# Autodesk Inventor assembly: SBGSMA6200ZZ-20
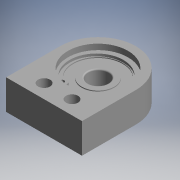
[picture p0: Inventor's stored thumbnail of the model, 180x180]
Saved by Autodesk Inventor 2017.3 (Build 213256000, 256)
## iProperties
Category: PARTsolutions
Company: MISUMI
Part Number: SBGSMA6200ZZ-20
Catalog Web Link: www.cadenas.de
Description: BGSMA, BGSMAB, SBGSMA-Bearing with Housings - Front Installation Type
Vendor: MISUMI
Document SubType Name: Assembly
Designer: partserver
Manufacturer: MISUMI
Mass: 18.5202 g
Surface Area: 96.0337 cm^2
Volume: 18.5202 cm^3
Density: 1 g/cm^3
Title: SBGSMA6200ZZ-20
Author: Cadenas PARTsolutions
Comments: Bearing with Housings - Front Installation Type
PSOL_IDENT_0: {$CADENAS_DATA\23d-libs\misumi\metric\12_bearing_holders\bgsma_asmtab.prj},222 {VTYP=3D},{STYP=ASSTA
PSOL_IDENT_1: B},{NB=SBGSMA6200ZZ-20},{LINA=SBGSMA6200ZZ-20},{NN=BGSMA, BGSMAB, SBGSMA},{DATE=09.09.2019 15:26:56}
PSOL_IDENT_2: ,{GEOMDATE=13.07.2015 10:17:28},{VERSION=},{LINEID=30},{WBVAR=MATB,STH,SEAL,HH,ALT1},{WBNUMERIC=HH}
PSOL_IDENT_3: {NB=SBGSMA6200ZZ-20},{LINA=SBGSMA6200ZZ-20},{KT=DUMMY},{PN=SBGSMA6200ZZ-20},{TYPE=SBGSMA},{MATB=STS
PSOL_IDENT_4: },{MATBALG= 'ST','Steel','STS','Stainless Steel' },{STH=},{STHALG= '','-' },{ARR=304 Stainless Steel
PSOL_IDENT_5: },{ARRALG=-S},{BN=6200},{SEAL=ZZ},{SEALALG= 'ZZ','ZZ(Double Shielded)','VV','VV(Non-contact Rubber S
PSOL_IDENT_6: eal)','DD','DD(Contact Rubber Seal)' },{HH=20},{HHALG=20,25,30},{DD=10},{D=30},{DDHH=24},{B=9},{H=46
PSOL_IDENT_7: .0},{HH1=7},{L=38},{L1=14},{T=15},{DD1=6},{ALT1=},{ALT1ALG= '','Bearing and Retaining Ring Assembled'
PSOL_IDENT_8: ,'NA','with NA (Bearing and Retaining Ring not Assembled)' },{ALT1PN=},{DD2=31.4},{TT=1.20},{PPATH=b
PSOL_IDENT_9: gsma/bgsma_asmtpl.prj}
NB: SBGSMA6200ZZ-20
NN: BGSMA, BGSMAB, SBGSMA
NT: Bearing with Housings - Front Installation Type
NBSYN: $PN.
LINA: SBGSMA6200ZZ-20
CATALOG: Misumi
PN: SBGSMA6200ZZ-20
MATB: Stainless Steel
STH: -
ARR: 304 Stainless Steel
BN: 6200
SEAL: ZZ(Double Shielded)
HH: 20
DD: 10
D: 30
DDHH: 24
B: 9
H: 46
HH1: 7
L: 38
L1: 14
T: 15
DD1: 6
ALT1: Bearing and Retaining Ring Assembled
SUPPLIER: MISUMI
ARTICLENO: SBGSMA6200ZZ-20
BOMINFO: SBGSMA6200ZZ-20
CREATOR: CADENAS GmbH
## Documents named in this file (4)
- e:\temp\worker_19\temp\exporttempdir_3676_132_Nk48c\format_0\SBGSMA6200ZZ-20.iam
- e:\temp\worker_19\temp\exporttempdir_3676_132_Nk48c\format_0\SBGSMA6200ZZ-20_h.ipt
- e:\temp\worker_19\temp\exporttempdir_3676_132_Nk48c\format_0\bearing_6200.ipt
- e:\temp\worker_19\temp\exporttempdir_3676_132_Nk48c\format_0\RRING-C-INT-S-30.ipt
## Components (3 placed, 3 different names)
1. SBGSMA6200ZZ-20_h:1 — to_bearing_XY@1 <-> center_point_XY@2, to_bearing_Z@1 <-> center_point_Z@2, to_bearing_YZ@1 <-> center_point_YZ@2, to_retaining_ring_XY@1 <-> rr_XY@3, to_retaining_ring_Z@1 <-> rr_Z@3, to_retaining_ring_YZ@1 <-> rr_YZ@3
2. bearing_6200:1 — to_bearing_XY@1 <-> center_point_XY@2, to_bearing_Z@1 <-> center_point_Z@2, to_bearing_YZ@1 <-> center_point_YZ@2
3. RRING-C-INT-S-30:1 — to_retaining_ring_XY@1 <-> rr_XY@3, to_retaining_ring_Z@1 <-> rr_Z@3, to_retaining_ring_YZ@1 <-> rr_YZ@3
## Relationships (6: Mate 4, Angle 2)
- to_bearing_XY@1 <-> center_point_XY@2 [Mate]: SBGSMA6200ZZ-20_h:1 ↔ bearing_6200:1
- to_bearing_Z@1 <-> center_point_Z@2 [Mate]: SBGSMA6200ZZ-20_h:1 ↔ bearing_6200:1
- to_bearing_YZ@1 <-> center_point_YZ@2 [Angle] (0 deg): SBGSMA6200ZZ-20_h:1 ↔ bearing_6200:1
- to_retaining_ring_XY@1 <-> rr_XY@3 [Mate]: SBGSMA6200ZZ-20_h:1 ↔ RRING-C-INT-S-30:1
- to_retaining_ring_Z@1 <-> rr_Z@3 [Mate]: SBGSMA6200ZZ-20_h:1 ↔ RRING-C-INT-S-30:1
- to_retaining_ring_YZ@1 <-> rr_YZ@3 [Angle] (0 deg): SBGSMA6200ZZ-20_h:1 ↔ RRING-C-INT-S-30:1
